# Autodesk Inventor assembly: servo_bottom_frame_with_nuts
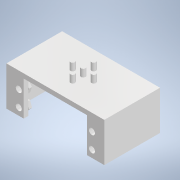
[picture p0: Inventor's stored thumbnail of the model, 180x180]
Saved by Autodesk Inventor 2021.4 (Build 254397000, 397)
## iProperties
Created: 2022-07-26
Part Number: servo_bottom_frame_with_nuts
Document SubType Name: Assembly
Designer: isamu
Author: isamu
## Documents named in this file (5)
- D:\personal_projects\robot\inventor\2021_matlab_compat _v2\servo_frames\servo_top_frame_with_nuts.iam
- D:\personal_projects\robot\exports\frames\servo frame with bottom.ipt
- D:\personal_projects\robot\exports\screws\m3x8.ipt
- D:\personal_projects\robot\exports\screws\m4x12.ipt
- D:\personal_projects\robot\exports\screws\m4 nuts.ipt
## Components (12 placed, 4 different names)
1. servo frame with bottom:1 — Insert:1, Insert:2, Insert:3, Insert:4, Insert:5, Insert:6, Insert:7, Insert:8, Insert:9, Insert:10, Insert:11
2. m3x8:1 — Insert:3
3. m3x8:2 — Insert:1
4. m3x8:3 — Insert:2
5. m3x8:4 — Insert:5
6. m3x8:5 — Insert:4
7. m4x12:1 — Insert:6
8. m4 nuts:1 — Insert:11
9. m4 nuts:2 — Insert:9
10. m4 nuts:3 — Insert:7
11. m4 nuts:4 — Insert:8
12. m4 nuts:5 — Insert:10
## Relationships (11: Insert 11)
- Insert:1: servo frame with bottom:1 ↔ m3x8:2
- Insert:2: servo frame with bottom:1 ↔ m3x8:3
- Insert:3: servo frame with bottom:1 ↔ m3x8:1
- Insert:4: servo frame with bottom:1 ↔ m3x8:5
- Insert:5: servo frame with bottom:1 ↔ m3x8:4
- Insert:6: servo frame with bottom:1 ↔ m4x12:1
- Insert:7: servo frame with bottom:1 ↔ m4 nuts:3
- Insert:8: servo frame with bottom:1 ↔ m4 nuts:4
- Insert:9: servo frame with bottom:1 ↔ m4 nuts:2
- Insert:10: servo frame with bottom:1 ↔ m4 nuts:5
- Insert:11: servo frame with bottom:1 ↔ m4 nuts:1
